# Autodesk Inventor assembly: SolenoidRack
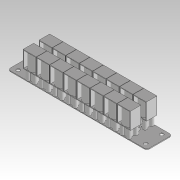
[picture p0: Inventor's stored thumbnail of the model, 180x180]
Saved by Autodesk Inventor 2020 (Build 240168000, 168)
## iProperties
Created: 2021-08-03
Part Number: SolenoidRack
Document SubType Name: Assembly
Designer: DDeGo
Author: DDeGo
## Documents named in this file (4)
- C:\Users\DDeGo\Documents\Drew\Projects\Gravity-Holo-Display\cad\SolenoidRack.iam
- C:\Users\DDeGo\Documents\Drew\Projects\Gravity-Holo-Display\cad\Solenoid.ipt
- C:\Users\DDeGo\Documents\Drew\Projects\Gravity-Holo-Display\cad\SolenoidBracket.ipt
- C:\Users\DDeGo\Documents\Drew\Projects\Gravity-Holo-Display\cad\SolenoidHead.ipt
## Components (33 placed, 3 different names)
1. SolenoidBracket:1 — Flush:1, Flush:2, Flush:3, Angle:1, Angle:2, Flush:4, Mate:5, Mate:6, Mate:13, Mate:14
2. SolenoidHead:2 — Mate:6, Mate:7, Mate:9, Mate:10, Mate:11, Mate:13
3. SolenoidHead:1 — Mate:5, Mate:8, Mate:9, Mate:12, Mate:14
4. Solenoid:2 — Angle:2, Mate:8, Mate:12
5. Solenoid:1 — Angle:1, Mate:7, Mate:10, Mate:11
6. SolenoidHead:3
7. SolenoidHead:4
8. Solenoid:3
9. Solenoid:4
10. SolenoidHead:5
11. SolenoidHead:6
12. Solenoid:5
13. Solenoid:6
14. SolenoidHead:7
15. SolenoidHead:8
16. Solenoid:7
17. Solenoid:8
18. SolenoidHead:9
19. SolenoidHead:10
20. Solenoid:9
21. Solenoid:10
22. SolenoidHead:11
23. SolenoidHead:12
24. Solenoid:11
25. Solenoid:12
26. SolenoidHead:13
27. SolenoidHead:14
28. Solenoid:13
29. Solenoid:14
30. SolenoidHead:15
31. SolenoidHead:16
32. Solenoid:15
33. Solenoid:16
## Component patterns: (8 elements, first: SolenoidHead:2 + SolenoidHead:1 + Solenoid:2 + Solenoid:1)
## Relationships (16: Mate 10, Flush 4, Angle 2)
- Flush:1: SolenoidBracket:1
- Flush:2: SolenoidBracket:1
- Flush:3: SolenoidBracket:1
- Angle:1 (0 deg): SolenoidBracket:1 ↔ Solenoid:1
- Angle:2 (0 deg): SolenoidBracket:1 ↔ Solenoid:2
- Flush:4: SolenoidBracket:1
- Mate:5: SolenoidBracket:1 ↔ SolenoidHead:1
- Mate:6: SolenoidBracket:1 ↔ SolenoidHead:2
- Mate:7: SolenoidHead:2 ↔ Solenoid:1
- Mate:8: SolenoidHead:1 ↔ Solenoid:2
- Mate:9: SolenoidHead:2 ↔ SolenoidHead:1
- Mate:10: SolenoidHead:2 ↔ Solenoid:1
- Mate:11: SolenoidHead:2 ↔ Solenoid:1
- Mate:12: SolenoidHead:1 ↔ Solenoid:2
- Mate:13: SolenoidBracket:1 ↔ SolenoidHead:2
- Mate:14: SolenoidBracket:1 ↔ SolenoidHead:1
